# Autodesk Inventor assembly: Complete back top housing
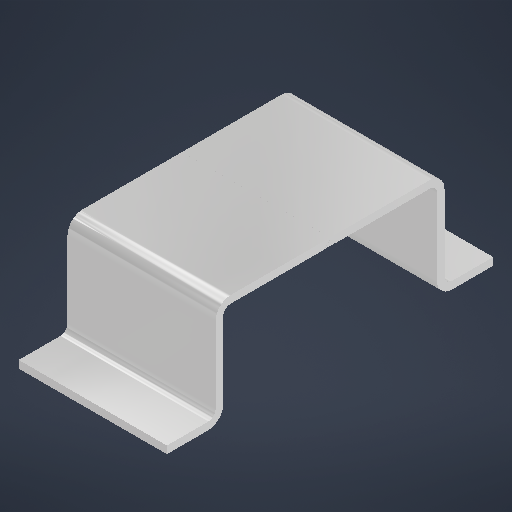
[picture p0: Inventor's stored thumbnail of the model, 512x512]
Saved by Autodesk Inventor 2026.3 (Build 303398000, 398)
## iProperties
Created: 2026-08-05
Part Number: Complete back top housing
Document SubType Name: Weldment
Designer: matot
Weld Material: Welded Aluminum-6061
Author: matot
## Documents named in this file (2)
- C:\Users\matot\OneDrive - Stellenbosch University\2026\MechatronicsProject478\Building the joint\Joint Assembly\Complete back top housing.iam
- C:\Users\matot\OneDrive - Stellenbosch University\2026\MechatronicsProject478\Building the joint\Joint Assembly\top front joint housing back.ipt
## Components (2 placed, 1 different names)
1. top front joint housing back:2 — Flush:1, Mate:1, Flush:2, Flush:3
2. top front joint housing back:3 — Flush:1, Mate:1, Flush:2, Flush:3
## Relationships (4: Flush 3, Mate 1)
- Flush:1: top front joint housing back:2 ↔ top front joint housing back:3
- Mate:1: top front joint housing back:2 ↔ top front joint housing back:3
- Flush:2: top front joint housing back:2 ↔ top front joint housing back:3
- Flush:3: top front joint housing back:2 ↔ top front joint housing back:3
